# Autodesk Inventor assembly: YPulleySupport
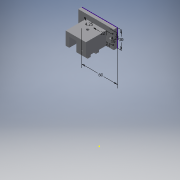
[picture p0: Inventor's stored thumbnail of the model, 180x180]
Saved by Autodesk Inventor 2019 (Build 230136000, 136)
## iProperties
Created: 2019-08-21
Part Number: YPulleySupport
Document SubType Name: Assembly
Designer: Bruno
Author: Bruno
## Documents named in this file (3)
- C:\Users\Bruno\Stuff\TPINFO\tp-info\YPulleySupport.iam
- C:\Users\Bruno\Stuff\TPINFO\tp-info\YPulleySupportBase.ipt
- C:\Users\Bruno\Stuff\TPINFO\tp-info\YPulleySupportHolder.ipt
## Components (2 placed, 2 different names)
1. YPulleySupportBase:1 — Mate:1, Cylindrical:1, Angle:1
2. YPulleySupportHolder:1 — Mate:1, Cylindrical:1, Angle:1
## Relationships (3: Mate 1, CylindricalJoint 1, Angle 1)
- Mate:1 (5 mm): YPulleySupportBase:1 ↔ YPulleySupportHolder:1
- Cylindrical:1: YPulleySupportBase:1 ↔ YPulleySupportHolder:1
- Angle:1 (0 deg): YPulleySupportBase:1 ↔ YPulleySupportHolder:1
